# Autodesk Inventor assembly: coincidenceCounter
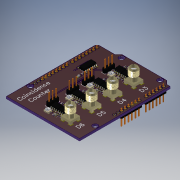
[picture p0: Inventor's stored thumbnail of the model, 180x180]
Saved by Autodesk Inventor 2016 (Build 200138000, 138)
## iProperties
Created: 2016-05-25
Part Number: coincidenceCounter
Document SubType Name: Assembly
Designer: Jonathan
Author: Jonathan
## Documents named in this file (15)
- C:\Users\Jonathan\Documents\Projects\nonmodular\coincidenceCounter\cad\coincidenceCounter.iam
- C:\Users\Jonathan\Documents\Projects\nonmodular\coincidenceCounter\cad\pcb.ipt
- C:\Users\Jonathan\Documents\Projects\nonmodular\coincidenceCounter\cad\electronics\soic\soic-14-N.ipt
- C:\Users\Jonathan\Documents\Projects\nonmodular\coincidenceCounter\cad\electronics\soic.ipt
- C:\Users\Jonathan\Documents\Projects\nonmodular\coincidenceCounter\cad\electronics\soic\soic-8-N.ipt
- C:\Users\Jonathan\Documents\Projects\nonmodular\coincidenceCounter\cad\electronics\CON-SMA001-SMG-G.ipt
- C:\Users\Jonathan\Documents\Projects\nonmodular\coincidenceCounter\cad\electronics\resistor\chipResistor\chipResistor-0402.ipt
- C:\Users\Jonathan\Documents\Projects\nonmodular\coincidenceCounter\cad\electronics\resistor\chipResistor.ipt
- C:\Users\Jonathan\Documents\Projects\nonmodular\coincidenceCounter\cad\electronics\PVZ3A\PVZ3A.iam
- C:\Users\Jonathan\Documents\Projects\nonmodular\coincidenceCounter\cad\electronics\capacitor\capacitor-0402.ipt
- C:\Users\Jonathan\Documents\Projects\nonmodular\coincidenceCounter\cad\electronics\capacitor\capacitor.ipt
- C:\Users\Jonathan\Documents\Projects\nonmodular\coincidenceCounter\cad\electronics\LTST-S270GKT.ipt
- C:\Users\Jonathan\Documents\Projects\nonmodular\coincidenceCounter\cad\electronics\2.54 breakaway\1x3.iam
- C:\Users\Jonathan\Documents\Projects\nonmodular\coincidenceCounter\cad\electronics\2.54 breakaway\1x8.iam
- C:\Users\Jonathan\Documents\Projects\nonmodular\coincidenceCounter\cad\electronics\2.54 breakaway\1x6.iam
## Components (72 placed, 11 different names)
1. pcb:1 — Mate:1, Angle:1, Angle:2, Angle:3, Angle:4, Angle:5, Angle:6, Angle:7, Angle:8, Angle:9, Mate:2, Mate:3, Mate:4, Flush:67, Mate:5, Angle:13, Angle:14, Angle:15, Angle:16, Mate:6, Mate:7, Mate:8, Mate:9, Mate:12, Mate:13, Angle:17, Angle:18, Angle:19, Angle:20, Angle:21, Mate:14, Mate:15, Mate:16, Mate:17, Mate:18, Mate:19
2. soic-14-N:1 — Flush:1, Mate:1, Angle:1
3. soic-8-N:2 — Flush:9, Angle:5, Flush:10
4. soic-8-N:3 — Flush:8, Flush:9, Angle:6, Flush:10
5. soic-8-N:4 — Flush:7, Flush:8, Angle:4, Flush:11
6. soic-8-N:5 — Flush:6, Flush:7, Angle:7, Flush:11
7. soic-8-N:6 — Flush:3, Flush:5, Flush:6, Angle:3, Flush:12
8. soic-8-N:7 — Flush:1, Flush:2, Flush:3, Flush:4, Flush:5, Angle:8, Flush:12
9. soic-8-N:8 — Flush:2, Angle:9, Flush:13
10. soic-8-N:9 — Flush:4, Angle:2, Flush:13
11. CON-SMA001-SMG-G:1 — Flush:14, Flush:16, Mate:2, Flush:19, Angle:22
12. CON-SMA001-SMG-G:2 — Flush:16, Flush:17, Flush:18
13. CON-SMA001-SMG-G:3 — Flush:14, Flush:15, Flush:18, Flush:19
14. CON-SMA001-SMG-G:4 — Flush:15, Flush:17
15. chipResistor-0402:6 — Flush:29, Angle:12, Flush:66
16. chipResistor-0402:7 — Angle:10, Flush:64
17. chipResistor-0402:8 — Flush:62, Angle:10, Angle:11, Flush:64, Flush:65, Flush:66
18. chipResistor-0402:10 — Flush:29, Flush:62, Angle:11, Angle:12, Flush:65, Flush:67
19. chipResistor-0402:14 — Flush:36
20. chipResistor-0402:15 — Flush:36
21. chipResistor-0402:16 — Flush:40
22. chipResistor-0402:17 — Flush:41, Flush:42
23. chipResistor-0402:18 — Flush:39
24. chipResistor-0402:20 — Flush:39, Flush:40, Flush:41
25. chipResistor-0402:21 — Flush:43, Mate:4
26. chipResistor-0402:22 — Flush:42, Flush:43, Flush:61
27. chipResistor-0402:23 — Flush:61
28. chipResistor-0402:25 — Flush:46, Flush:47, Flush:48
29. chipResistor-0402:26 — Flush:47, Flush:50, Flush:55
30. chipResistor-0402:27 — Flush:54
31. chipResistor-0402:28 — Flush:49, Mate:5, Flush:70, Angle:13
32. chipResistor-0402:29 — Flush:46, Flush:49
33. chipResistor-0402:30 — Flush:48, Flush:55
34. chipResistor-0402:31 — Flush:51, Flush:54
35. chipResistor-0402:32 — Flush:50, Flush:51, Flush:52
36. chipResistor-0402:33 — Flush:52, Flush:53
37. chipResistor-0402:34 — Flush:53, Flush:56
38. chipResistor-0402:35 — Flush:57
39. chipResistor-0402:36 — Flush:63
40. chipResistor-0402:38 — Flush:59
41. chipResistor-0402:39 — Flush:56, Flush:57, Flush:58
42. chipResistor-0402:40 — Flush:58, Flush:59, Flush:63
43. PVZ3A:1 [sub-assembly] — Flush:21, Flush:22
44. PVZ3A:2 [sub-assembly] — Flush:20, Flush:21
45. PVZ3A:3 [sub-assembly] — Flush:22
46. PVZ3A:4 [sub-assembly] — Flush:20, Mate:3
47. chipResistor-0402:41 — Flush:68, Angle:14
48. chipResistor-0402:42 — Flush:69, Flush:70, Angle:15
49. chipResistor-0402:43 — Flush:68, Flush:69, Angle:16
50. chipResistor-0402:44 — Mate:6
51. capacitor-0402:1 — Flush:71, Flush:72
52. capacitor-0402:2 — Flush:71, Mate:7
53. capacitor-0402:3 — Flush:72, Flush:73
54. capacitor-0402:4 — Flush:73
55. capacitor-0402:5 — Flush:74
56. capacitor-0402:6 — Flush:74, Flush:75
57. capacitor-0402:7 — Flush:75, Flush:76, Mate:8
58. capacitor-0402:8 — Flush:76
59. chipResistor-0402:45 — Mate:9
60. LTST-S270GKT:1 — Flush:79, Mate:13, Angle:17
61. LTST-S270GKT:2 — Flush:77, Flush:78, Angle:20
62. LTST-S270GKT:3 — Flush:78, Flush:79, Mate:12, Angle:18
63. LTST-S270GKT:4 — Angle:21, Mate:14
64. LTST-S270GKT:5 — Flush:77, Angle:19
65. 1x3:1 [sub-assembly] — Mate:15, Angle:22, Flush:80
66. 1x3:2 [sub-assembly] — Flush:80, Flush:81
67. 1x3:3 [sub-assembly] — Flush:81, Flush:82
68. 1x3:4 [sub-assembly] — Flush:82
69. 1x8:1 [sub-assembly] — Mate:16
70. 1x8:2 [sub-assembly] — Mate:17
71. 1x6:1 [sub-assembly] — Mate:19
72. 1x6:2 [sub-assembly] — Mate:18
## Relationships (104: Flush 65, Angle 22, Mate 17)
- Flush:1: soic-14-N:1 ↔ soic-8-N:7
- Flush:2: soic-8-N:7 ↔ soic-8-N:8
- Flush:3: soic-8-N:6 ↔ soic-8-N:7
- Flush:4: soic-8-N:7 ↔ soic-8-N:9
- Flush:5: soic-8-N:6 ↔ soic-8-N:7
- Flush:6: soic-8-N:5 ↔ soic-8-N:6
- Flush:7: soic-8-N:4 ↔ soic-8-N:5
- Flush:8: soic-8-N:3 ↔ soic-8-N:4
- Flush:9: soic-8-N:2 ↔ soic-8-N:3
- Mate:1: pcb:1 ↔ soic-14-N:1
- Angle:1 (0 deg): pcb:1 ↔ soic-14-N:1
- Angle:2 (0 deg): pcb:1 ↔ soic-8-N:9
- Angle:3 (0 deg): pcb:1 ↔ soic-8-N:6
- Angle:4 (0 deg): pcb:1 ↔ soic-8-N:4
- Angle:5 (0 deg): pcb:1 ↔ soic-8-N:2
- Angle:6 (0 deg): pcb:1 ↔ soic-8-N:3
- Angle:7 (0 deg): pcb:1 ↔ soic-8-N:5
- Angle:8 (0 deg): pcb:1 ↔ soic-8-N:7
- Angle:9 (0 deg): pcb:1 ↔ soic-8-N:8
- Flush:10: soic-8-N:2 ↔ soic-8-N:3
- Flush:11: soic-8-N:4 ↔ soic-8-N:5
- Flush:12: soic-8-N:6 ↔ soic-8-N:7
- Flush:13: soic-8-N:8 ↔ soic-8-N:9
- Flush:14: CON-SMA001-SMG-G:1 ↔ CON-SMA001-SMG-G:3
- Flush:15: CON-SMA001-SMG-G:3 ↔ CON-SMA001-SMG-G:4
- Flush:16: CON-SMA001-SMG-G:1 ↔ CON-SMA001-SMG-G:2
- Mate:2: pcb:1 ↔ CON-SMA001-SMG-G:1
- Flush:17: CON-SMA001-SMG-G:2 ↔ CON-SMA001-SMG-G:4
- Flush:18: CON-SMA001-SMG-G:2 ↔ CON-SMA001-SMG-G:3
- Flush:19: CON-SMA001-SMG-G:1 ↔ CON-SMA001-SMG-G:3
- Flush:20: PVZ3A:2 ↔ PVZ3A:4
- Flush:21: PVZ3A:1 ↔ PVZ3A:2
- Flush:22: PVZ3A:1 ↔ PVZ3A:3
- Mate:3: pcb:1 ↔ PVZ3A:4
- Flush:29: chipResistor-0402:6 ↔ chipResistor-0402:10
- Flush:36: chipResistor-0402:14 ↔ chipResistor-0402:15
- Flush:39: chipResistor-0402:18 ↔ chipResistor-0402:20
- Flush:40: chipResistor-0402:16 ↔ chipResistor-0402:20
- Flush:41: chipResistor-0402:17 ↔ chipResistor-0402:20
- Flush:42: chipResistor-0402:17 ↔ chipResistor-0402:22
- Flush:43: chipResistor-0402:21 ↔ chipResistor-0402:22
- Flush:46: chipResistor-0402:25 ↔ chipResistor-0402:29
- Flush:47: chipResistor-0402:25 ↔ chipResistor-0402:26
- Flush:48: chipResistor-0402:25 ↔ chipResistor-0402:30
- Flush:49: chipResistor-0402:28 ↔ chipResistor-0402:29
- Flush:50: chipResistor-0402:26 ↔ chipResistor-0402:32
- Flush:51: chipResistor-0402:31 ↔ chipResistor-0402:32
- Flush:52: chipResistor-0402:32 ↔ chipResistor-0402:33
- Flush:53: chipResistor-0402:33 ↔ chipResistor-0402:34
- Flush:54: chipResistor-0402:27 ↔ chipResistor-0402:31
- Flush:55: chipResistor-0402:26 ↔ chipResistor-0402:30
- Flush:56: chipResistor-0402:34 ↔ chipResistor-0402:39
- Flush:57: chipResistor-0402:35 ↔ chipResistor-0402:39
- Flush:58: chipResistor-0402:39 ↔ chipResistor-0402:40
- Flush:59: chipResistor-0402:38 ↔ chipResistor-0402:40
- Flush:61: chipResistor-0402:22 ↔ chipResistor-0402:23
- Flush:62: chipResistor-0402:8 ↔ chipResistor-0402:10
- Flush:63: chipResistor-0402:36 ↔ chipResistor-0402:40
- Mate:4: pcb:1 ↔ chipResistor-0402:21
- Angle:10 (0 deg): chipResistor-0402:7 ↔ chipResistor-0402:8
- Angle:11 (0 deg): chipResistor-0402:8 ↔ chipResistor-0402:10
- Angle:12 (0 deg): chipResistor-0402:6 ↔ chipResistor-0402:10
- Flush:64: chipResistor-0402:7 ↔ chipResistor-0402:8
- Flush:65: chipResistor-0402:8 ↔ chipResistor-0402:10
- Flush:66: chipResistor-0402:6 ↔ chipResistor-0402:8
- Flush:67: pcb:1 ↔ chipResistor-0402:10
- Mate:5: pcb:1 ↔ chipResistor-0402:28
- Flush:68: chipResistor-0402:41 ↔ chipResistor-0402:43
- Flush:69: chipResistor-0402:42 ↔ chipResistor-0402:43
- Flush:70: chipResistor-0402:28 ↔ chipResistor-0402:42
- Angle:13 (0 deg): pcb:1 ↔ chipResistor-0402:28
- Angle:14 (0 deg): pcb:1 ↔ chipResistor-0402:41
- Angle:15 (0 deg): pcb:1 ↔ chipResistor-0402:42
- Angle:16 (0 deg): pcb:1 ↔ chipResistor-0402:43
- Mate:6: pcb:1 ↔ chipResistor-0402:44
- Flush:71: capacitor-0402:1 ↔ capacitor-0402:2
- Flush:72: capacitor-0402:1 ↔ capacitor-0402:3
- Flush:73: capacitor-0402:3 ↔ capacitor-0402:4
- Mate:7: pcb:1 ↔ capacitor-0402:2
- Flush:74: capacitor-0402:5 ↔ capacitor-0402:6
- Flush:75: capacitor-0402:6 ↔ capacitor-0402:7
- Flush:76: capacitor-0402:7 ↔ capacitor-0402:8
- Mate:8: pcb:1 ↔ capacitor-0402:7
- Mate:9: pcb:1 ↔ chipResistor-0402:45
- Flush:77: LTST-S270GKT:2 ↔ LTST-S270GKT:5
- Flush:78: LTST-S270GKT:2 ↔ LTST-S270GKT:3
- Flush:79: LTST-S270GKT:1 ↔ LTST-S270GKT:3
- Mate:12: pcb:1 ↔ LTST-S270GKT:3
- Mate:13: pcb:1 ↔ LTST-S270GKT:1
- Angle:17 (0 deg): pcb:1 ↔ LTST-S270GKT:1
- Angle:18 (0 deg): pcb:1 ↔ LTST-S270GKT:3
- Angle:19 (0 deg): pcb:1 ↔ LTST-S270GKT:5
- Angle:20 (0 deg): pcb:1 ↔ LTST-S270GKT:2
- Angle:21 (0 deg): pcb:1 ↔ LTST-S270GKT:4
- Mate:14: pcb:1 ↔ LTST-S270GKT:4
- Mate:15: pcb:1 ↔ 1x3:1
- Angle:22 (0 deg): CON-SMA001-SMG-G:1 ↔ 1x3:1
- Flush:80: 1x3:1 ↔ 1x3:2
- Flush:81: 1x3:2 ↔ 1x3:3
- Flush:82: 1x3:3 ↔ 1x3:4
- Mate:16: pcb:1 ↔ 1x8:1
- Mate:17: pcb:1 ↔ 1x8:2
- Mate:18: pcb:1 ↔ 1x6:2
- Mate:19: pcb:1 ↔ 1x6:1
